# Autodesk Inventor assembly: Center Assembly
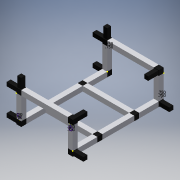
[picture p0: Inventor's stored thumbnail of the model, 180x180]
Saved by Autodesk Inventor 2017 (Build 210142000, 142)
## iProperties
Created: 2019-12-06
Part Number: Center Assembly
Document SubType Name: Assembly
Designer: S346553810
Author: S346553810
## Documents named in this file (9)
- \\ad.ocdsb.ca\studenthome\3\S338674153\FRC 2020\FullRobotRefactor\SubFrame\Center Assembly.iam
- \\ad.ocdsb.ca\studenthome\3\S338674153\FRC 2020\FullRobotRefactor\SubFrame\center cross-member.iam
- \\ad.ocdsb.ca\studenthome\3\S338674153\FRC 2020\FullRobotRefactor\SubFrame\1in sq tub - 4.ipt
- \\ad.ocdsb.ca\studenthome\3\S338674153\FRC 2020\FullRobotRefactor\SubFrame\Kipp K0617.ipt
- \\ad.ocdsb.ca\studenthome\3\S338674153\FRC 2020\FullRobotRefactor\SubFrame\Kipp K0619.ipt
- \\ad.ocdsb.ca\studenthome\3\S338674153\FRC 2020\FullRobotRefactor\SubFrame\1in sq tub - 6.ipt
- \\ad.ocdsb.ca\studenthome\3\S338674153\FRC 2020\FullRobotRefactor\SubFrame\1in sq tub - 4-5.ipt
- \\ad.ocdsb.ca\studenthome\3\S338674153\FRC 2020\FullRobotRefactor\SubFrame\1in sq tub - 6-5.ipt
- \\ad.ocdsb.ca\studenthome\3\S338674153\FRC 2020\FullRobotRefactor\KIPS\Kipp K0618.ipt
## Components (14 placed, 8 different names)
1. center cross-member:1 [sub-assembly] — Mate:15, Mate:16, Mate:17, Mate:18, Mate:19, Mate:20, Flush:8, Flush:13
2. 1in sq tub - 4:1 — Mate:9, Mate:10, Mate:11
3. 1in sq tub - 4:2 — Mate:21, Mate:22, Mate:23, Mate:24, Flush:5, Mate:25
4. Kipp K0617:1 — Mate:5, Mate:6, Mate:7
5. Kipp K0617:2 — Mate:3, Mate:4, Mate:8, Mate:21, Mate:22, Mate:23
6. Kipp K0619:1 — Mate:24, Flush:5, Mate:25, Mate:26, Mate:27, Mate:28
7. Kipp K0619:2 — Mate:9, Mate:10, Mate:11, Mate:12, Mate:13, Mate:14
8. 1in sq tub - 6:1 — Mate:15, Mate:16, Mate:17
9. 1in sq tub - 4-5:1 — Mate:26, Mate:27, Mate:28, Flush:6, Flush:7
10. 1in sq tub - 4-5:2 — Mate:12, Mate:13, Mate:14, Flush:9, Flush:10
11. 1in sq tub - 6:3 — Mate:18, Mate:19, Mate:20, Flush:11, Flush:12, Flush:13
12. 1in sq tub - 6-5:1 — Mate:3, Mate:4, Mate:5, Mate:6, Mate:7, Mate:8
13. Kipp K0618:1 — Flush:9, Flush:10, Flush:11, Flush:12
14. Kipp K0618:2 — Flush:6, Flush:7, Flush:8
## Relationships (41: Mate 28, Flush 13)
- [Mate]: Kipp K0617:1 ↔ 1in sq tub - 6:1
- [Flush]: Kipp K0617:1 ↔ 1in sq tub - 6:1
- [Flush]: Kipp K0617:1 ↔ 1in sq tub - 6:1
- [Mate]: 1in sq tub - 4:1 ↔ Kipp K0617:1
- [Flush]: 1in sq tub - 4:1 ↔ Kipp K0617:1
- [Flush]: 1in sq tub - 4:1 ↔ Kipp K0617:1
- Mate:3: Kipp K0617:2 ↔ 1in sq tub - 6-5:1
- Mate:4: Kipp K0617:2 ↔ 1in sq tub - 6-5:1
- Mate:5: Kipp K0617:1 ↔ 1in sq tub - 6-5:1
- Mate:6: Kipp K0617:1 ↔ 1in sq tub - 6-5:1
- Mate:7: Kipp K0617:1 ↔ 1in sq tub - 6-5:1
- Mate:8: Kipp K0617:2 ↔ 1in sq tub - 6-5:1
- Mate:9: 1in sq tub - 4:1 ↔ Kipp K0619:2
- Mate:10: 1in sq tub - 4:1 ↔ Kipp K0619:2
- Mate:11: 1in sq tub - 4:1 ↔ Kipp K0619:2
- Mate:12: Kipp K0619:2 ↔ 1in sq tub - 4-5:2
- Mate:13: Kipp K0619:2 ↔ 1in sq tub - 4-5:2
- Mate:14: Kipp K0619:2 ↔ 1in sq tub - 4-5:2
- Mate:15: center cross-member:1 ↔ 1in sq tub - 6:1
- Mate:16: center cross-member:1 ↔ 1in sq tub - 6:1
- Mate:17: center cross-member:1 ↔ 1in sq tub - 6:1
- Mate:18: center cross-member:1 ↔ 1in sq tub - 6:3
- Mate:19: center cross-member:1 ↔ 1in sq tub - 6:3
- Mate:20: center cross-member:1 ↔ 1in sq tub - 6:3
- Mate:21: 1in sq tub - 4:2 ↔ Kipp K0617:2
- Mate:22: 1in sq tub - 4:2 ↔ Kipp K0617:2
- Mate:23: 1in sq tub - 4:2 ↔ Kipp K0617:2
- Mate:24: 1in sq tub - 4:2 ↔ Kipp K0619:1
- Flush:5: 1in sq tub - 4:2 ↔ Kipp K0619:1
- Mate:25: 1in sq tub - 4:2 ↔ Kipp K0619:1
- Mate:26: Kipp K0619:1 ↔ 1in sq tub - 4-5:1
- Mate:27: Kipp K0619:1 ↔ 1in sq tub - 4-5:1
- Mate:28: Kipp K0619:1 ↔ 1in sq tub - 4-5:1
- Flush:6: 1in sq tub - 4-5:1 ↔ Kipp K0618:2
- Flush:7: 1in sq tub - 4-5:1 ↔ Kipp K0618:2
- Flush:8: center cross-member:1 ↔ Kipp K0618:2
- Flush:9: 1in sq tub - 4-5:2 ↔ Kipp K0618:1
- Flush:10: 1in sq tub - 4-5:2 ↔ Kipp K0618:1
- Flush:11: 1in sq tub - 6:3 ↔ Kipp K0618:1
- Flush:12: 1in sq tub - 6:3 ↔ Kipp K0618:1
- Flush:13: center cross-member:1 ↔ 1in sq tub - 6:3
## Named parameters: d5_d7 = 0 mm, d6_d8 = 0 mm, d7_d9 = 0 mm, d8_d10 = 0 mm
